# Autodesk Inventor assembly: odomPods
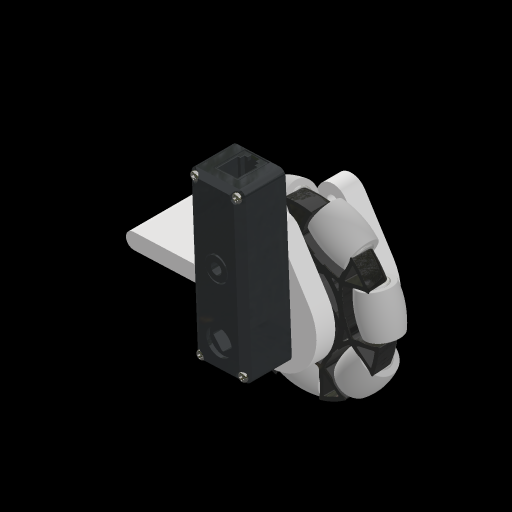
[picture p0: Inventor's stored thumbnail of the model, 512x512]
Saved by Autodesk Inventor 2024.1 (Build 281209000, 209)
## iProperties
Created: 2025-05-24
Part Number: odomPods
Document SubType Name: Assembly
Designer: Teddy
Author: Teddy
## Documents named in this file (4)
- C:\Users\Teddy\OneDrive\Desktop\VEX-CAD-Inventor-1.4.0\pushBack\PushBackBot2\odomPods.iam
- C:\Users\Teddy\OneDrive\Desktop\VEX-CAD-Inventor-1.4.0\Motion\Wheels\Omni Wheel\2.75 Omni Half.ipt
- C:\Users\Teddy\OneDrive\Desktop\VEX-CAD-Inventor-1.4.0\Electronics\Sensors\V5 Rotation Sensor.ipt
- C:\Users\Teddy\OneDrive\Desktop\VEX-CAD-Inventor-1.4.0\pushBack\PushBackBot2\odomHousing.ipt
## Components (3 placed, 3 different names)
1. V5 Rotation Sensor:1 — Insert:2, Insert:3
2. odomHousing:1 — Insert:1, Insert:2, Insert:3
3. 2.75 Omni Half:1 — Insert:1
## Relationships (3: Insert 3)
- Insert:1 (3.81 mm): odomHousing:1 ↔ 2.75 Omni Half:1
- Insert:2: V5 Rotation Sensor:1 ↔ odomHousing:1
- Insert:3: V5 Rotation Sensor:1 ↔ odomHousing:1
